# Autodesk Inventor assembly: wheel1
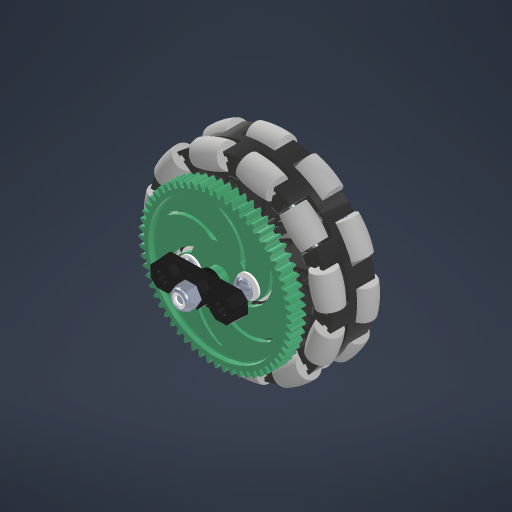
[picture p0: Inventor's stored thumbnail of the model, 512x512]
Saved by Autodesk Inventor 2024 (Build 280153000, 153)
## iProperties
Created: 2023-08-09
Part Number: wheel1
Document SubType Name: Assembly
Designer: macbook
Author: macbook
## Documents named in this file (18)
- \\Mac\Home\Desktop\code\1599V-VRC\Cad\Assembly\v2\omniwheel.iam
- \\Mac\Home\Desktop\code\1599V-VRC\Cad\Motion\Shaft LS\Bearing Flat.ipt
- \\Mac\Home\Desktop\code\1599V-VRC\Cad\Motion\Spacers\Washer Teflon\TWasher .375 OD x .03125.ipt
- \\Mac\Home\Desktop\code\1599V-VRC\Cad\Structure\Hardware\Nut Nylock.ipt
- \\Mac\Home\Desktop\code\1599V-VRC\Cad\Structure\Hardware\Screw Steel - Star\SScrew Star Smooth 2.500.ipt
- \\Mac\Home\Desktop\code\1599V-VRC\Cad\Motion\Gears\LS 60T Gear.ipt
- \\Mac\Home\Desktop\code\1599V-VRC\Cad\Structure\Hardware\Screw Steel - Star\SScrew Star Threaded 1.250.ipt
- \\Mac\Home\Desktop\code\1599V-VRC\Cad\Motion\Spacers\Spacer Nylon .500 OD\NSpacer White .500 OD x .375.ipt
- \\Mac\Home\Desktop\code\1599V-VRC\Cad\Motion\Spacers\Washer Steel\SWasher .375 OD x .015625.ipt
- \\Mac\Home\Desktop\code\1599V-VRC\Cad\Motion\Spacers\Spacer Nylon .500 OD\NSpacer White .500 OD x .500.ipt
- \\Mac\Home\Desktop\code\1599V-VRC\Cad\Motion\Spacers\Spacer Nylon Click On\Nspacer Click On x .1250.ipt
- \\Mac\Home\Desktop\code\1599V-VRC\Cad\Motion\Spacers\Spacer Nylon Click On.ipt
- \\Mac\Home\Desktop\code\1599V-VRC\Cad\Motion\Wheels\Omni Wheel\3.25 Omni AS, cir.iam
- \\Mac\Home\Desktop\code\1599V-VRC\Cad\Motion\Spacers\Spacer Nylon Click On\Nspacer Click On x .0625.ipt
- \\Mac\Home\Desktop\code\1599V-VRC\Cad\Structure\Hardware\Screw Steel - Star.ipt
- \\Mac\Home\Desktop\code\1599V-VRC\Cad\Motion\Spacers\Spacer Nylon .500 OD.ipt
- \\Mac\Home\Desktop\code\1599V-VRC\Cad\Motion\Spacers\Washer Steel.ipt
- \\Mac\Home\Desktop\code\1599V-VRC\Cad\Motion\Spacers\Washer Teflon.ipt
## Components (18 placed, 12 different names)
1. 3.25 Omni AS, cir:1 [sub-assembly] — Insert:92, Insert:94, Insert:95, Insert:97
2. Nspacer Click On x .1250:1 — Insert:98
3. Bearing Flat:2 — Insert:46, Insert:47, Insert:71
4. Bearing Flat:3 — Insert:46, Insert:47, Insert:70, Insert:99
5. LS 60T Gear:1 — Insert:82, Insert:84, Insert:86, Insert:91, Insert:98
6. SScrew Star Threaded 1.250:11 — Insert:83, Rotational:1
7. Nut Nylock:4 — Insert:94, Rotational:1
8. Nut Nylock:5 — Insert:97
9. SScrew Star Threaded 1.250:12 — Insert:85
10. SScrew Star Smooth 2.500:14 — Insert:70
11. Nut Nylock:6 — Insert:71
12. NSpacer White .500 OD x .500:5 — Insert:95, Insert:96
13. SWasher .375 OD x .015625:2 — Insert:81, Insert:82
14. NSpacer White .500 OD x .375:6 — Insert:81
15. TWasher .375 OD x .03125:9 — Insert:83, Insert:84
16. TWasher .375 OD x .03125:10 — Insert:85, Insert:86
17. Nspacer Click On x .0625:2 — Insert:96, Insert:99
18. NSpacer White .500 OD x .375:7 — Insert:91, Insert:92
## Relationships (22: Insert 21, RevoluteJoint 1)
- [Insert] (1.5875 mm): Nspacer Click On x .1250:1 ↔ Bearing Flat:2
- Insert:46 (44.45 mm): Bearing Flat:2 ↔ Bearing Flat:3
- Insert:47 (44.45 mm): Bearing Flat:2 ↔ Bearing Flat:3
- [Insert]: Nspacer Click On x .1250:1 ↔ LS 60T Gear:1
- Insert:70 (1.5875 mm): Bearing Flat:3 ↔ SScrew Star Smooth 2.500:14
- Insert:71: Bearing Flat:2 ↔ Nut Nylock:6
- Insert:81: SWasher .375 OD x .015625:2 ↔ NSpacer White .500 OD x .375:6
- Insert:82: LS 60T Gear:1 ↔ SWasher .375 OD x .015625:2
- Insert:83: SScrew Star Threaded 1.250:11 ↔ TWasher .375 OD x .03125:9
- Insert:84: LS 60T Gear:1 ↔ TWasher .375 OD x .03125:9
- Insert:85: SScrew Star Threaded 1.250:12 ↔ TWasher .375 OD x .03125:10
- Insert:86: LS 60T Gear:1 ↔ TWasher .375 OD x .03125:10
- Insert:91: LS 60T Gear:1 ↔ NSpacer White .500 OD x .375:7
- Insert:92: 3.25 Omni AS, cir:1 ↔ NSpacer White .500 OD x .375:7
- [Insert]: NSpacer White .500 OD x .500:5 ↔ Nspacer Click On x .0625:2
- Insert:94: 3.25 Omni AS, cir:1 ↔ Nut Nylock:4
- Insert:95: 3.25 Omni AS, cir:1 ↔ NSpacer White .500 OD x .500:5
- Insert:96: NSpacer White .500 OD x .500:5 ↔ Nspacer Click On x .0625:2
- Insert:97: 3.25 Omni AS, cir:1 ↔ Nut Nylock:5
- Rotational:1 [RevoluteJoint]: SScrew Star Threaded 1.250:11 ↔ Nut Nylock:4
- Insert:98: Nspacer Click On x .1250:1 ↔ LS 60T Gear:1
- Insert:99: Bearing Flat:3 ↔ Nspacer Click On x .0625:2
